# Autodesk Inventor assembly: board_setter
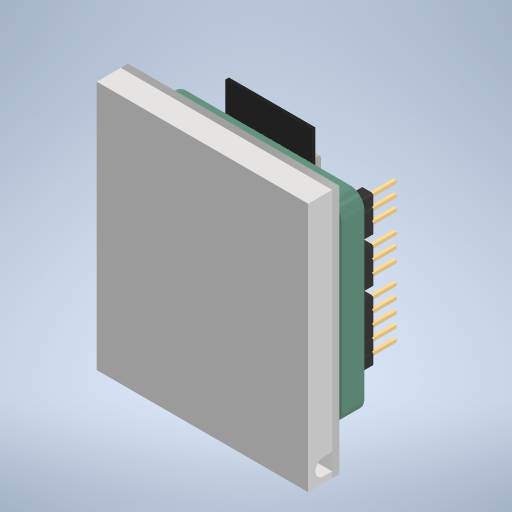
[picture p0: Inventor's stored thumbnail of the model, 512x512]
Saved by Autodesk Inventor 2024.1 (Build 281209000, 209)
## iProperties
Created: 2024-10-09
Part Number: board_setter
Document SubType Name: Assembly
Designer: hibik
Author: hibik
## Documents named in this file (4)
- C:\Users\hibik\Documents\Robomech\HR\Eglantyne\hard\upper_body\chest\board_setter.iam
- C:\Users\hibik\Documents\Robomech\HR\Eglantyne\hard\upper_body\chest\board_setter_base.ipt
- C:\Users\hibik\Documents\Robomech\HR\Eglantyne\hard\upper_body\chest\board_setter_cover.ipt
- C:\Users\hibik\Documents\Robomech\HR\Eglantyne\hard\needed_model\ControlBoard.iam
## Components (3 placed, 3 different names)
1. board_setter_base:1 — 挿入:1, 挿入:2
2. board_setter_cover:1 — 挿入:1, 挿入:2, 挿入:3, 挿入:4
3. ControlBoard:1 [sub-assembly] — 挿入:3, 挿入:4
## Relationships (4: Insert 4)
- 挿入:1 [Insert]: board_setter_base:1 ↔ board_setter_cover:1
- 挿入:2 [Insert]: board_setter_base:1 ↔ board_setter_cover:1
- 挿入:3 [Insert]: board_setter_cover:1 ↔ ControlBoard:1
- 挿入:4 [Insert]: board_setter_cover:1 ↔ ControlBoard:1
